# Autodesk Inventor assembly: ABD_Version_0.1_leftleg
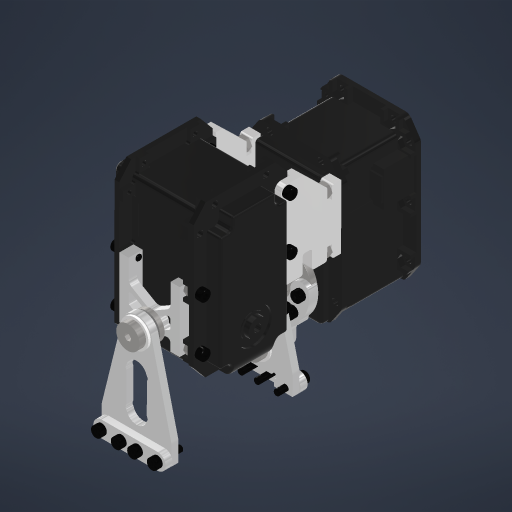
[picture p0: Inventor's stored thumbnail of the model, 512x512]
Saved by Autodesk Inventor 2024.3 (Build 283343000, 343)
## iProperties
Created: 2024-01-23
Part Number: ABD_Version_0.1_leftleg
Document SubType Name: Assembly
Designer: ASUS
Mass: 357.136 g
Surface Area: 604.848 cm^2
Volume: 181.423 cm^3
Density: 1.96853 g/cm^3
Author: ASUS
## Documents named in this file (19)
- C:\Users\ASUS\Desktop\test\v4_Frame\ABD_V4_Left_OP.iam
- C:\Users\ASUS\Desktop\test\v4_Frame\ABD_MX_64_Roll_Fixation_Set.iam
- C:\Users\ASUS\Desktop\test\v4_Frame\ABD_Slider_Set_v4.iam
- C:\Users\ASUS\Desktop\test\v1_Frame\MISUMI\C-WSSA12-4-2.ipt
- C:\Users\ASUS\Desktop\test\v4_Frame\Roll_Fixation_Frame_Back.ipt
- C:\Users\ASUS\Desktop\test\v4_Frame\hip joint fix washer.ipt
- C:\Users\ASUS\Desktop\test\Screw_Set\hip_joint_fix_washer_10mm_Set.iam
- C:\Users\ASUS\Desktop\test\v4_Frame\Front_Frame_Fixer_v2.iam
- C:\Users\ASUS\Desktop\test\ROBOTIS(Inventor 2024 ver.)\DXL\MX-64T.ipt
- C:\Users\ASUS\Desktop\test\v2_Frame\MISUMI\DBSY4-5-8.ipt
- C:\Users\ASUS\Desktop\test\v4_Frame\Dynamixel Vertical fixation.ipt
- C:\Users\ASUS\Desktop\test\v4_Frame\Dynamixel Vertical fixation_MIR.ipt
- C:\Users\ASUS\Desktop\test\v1_Frame\MISUMI\SLBNR2_5.ipt
- C:\Users\ASUS\Desktop\test\v4_Frame\MISUMI\TT-0612-05.ipt
- C:\Users\ASUS\Desktop\test\v4_Frame\MISUMI\LED-0605.ipt
- C:\Users\ASUS\Desktop\test\v4_Frame\MISUMI\DBB4-6-6.ipt
- C:\Users\ASUS\Desktop\test\v4_Frame\MISUMI\DBGS4-5-8.ipt
- C:\Users\ASUS\Desktop\test\Screw_Set\Roll_Fixation_Frame_8mm_Set.iam
- C:\Users\ASUS\Desktop\test\Screw_Set\Roll_Fixation_Frame_8mm_Set_Backside.iam
## Components (26 placed, 18 different names)
1. hip joint fix washer:1 — 삽입:64
2. hip joint fix washer:2 — 삽입:47, 메이트:29
3. hip_joint_fix_washer_10mm_Set:1 [sub-assembly] — 메이트:39
4. hip_joint_fix_washer_10mm_Set:2 [sub-assembly] — 메이트:29, 메이트:43
5. Front_Frame_Fixer_v2:1 [sub-assembly] — 삽입:46, 삽입:63, 삽입:73
6. DBSY4-5-8:1 — 삽입:73
7. ABD_MX_64_Roll_Fixation_Set:2 [sub-assembly] — 각도:3, 플러쉬:1, 삽입:46, 삽입:52, 삽입:71, 메이트:45, 삽입:72, 메이트:46
8. MX-64T:1 — 삽입:43, 각도:3, 플러쉬:1, 삽입:61, 메이트:35, 삽입:62, 메이트:36, 각도:13
9. ABD_Slider_Set_v4:2 [sub-assembly] — 삽입:43, 삽입:69
10. Roll_Fixation_Frame_Back:3 — 삽입:47, 메이트:43, 삽입:68, 메이트:44, 각도:13
11. Front_Frame_Fixer_v2:2 [sub-assembly] — 삽입:52, 삽입:68, 삽입:70
12. Dynamixel Vertical fixation:2 — 삽입:61, 메이트:35, 메이트:47, 메이트:48
13. Dynamixel Vertical fixation_MIR:2 — 삽입:62, 메이트:36
14. SLBNR2_5:5
15. SLBNR2_5:6
16. SLBNR2_5:7
17. SLBNR2_5:8
18. Roll_Fixation_Frame_Back:4 — 삽입:63, 메이트:39, 삽입:64
19. C-WSSA12-4-2:3 — 삽입:69
20. TT-0612-05:1
21. TT-0612-05:2
22. LED-0605:1 — 메이트:44
23. DBB4-6-6:1
24. DBGS4-5-8:1 — 삽입:70
25. Roll_Fixation_Frame_8mm_Set:1 [sub-assembly] — 삽입:71, 메이트:45
26. Roll_Fixation_Frame_8mm_Set_Backside:1 [sub-assembly] — 삽입:72, 메이트:46, 메이트:47, 메이트:48
## Relationships (46: Insert 23, Mate 16, Angle 6, Flush 1)
- [Insert]: hip joint fix washer:1 ↔ hip_joint_fix_washer_10mm_Set:1
- [Mate]: hip joint fix washer:1 ↔ hip_joint_fix_washer_10mm_Set:1
- [Insert]: hip joint fix washer:2 ↔ hip_joint_fix_washer_10mm_Set:2
- [Mate]: hip joint fix washer:2 ↔ hip_joint_fix_washer_10mm_Set:2
- [Mate]: hip_joint_fix_washer_10mm_Set:1 ↔ hip_joint_fix_washer_10mm_Set:2
- [Mate]: hip_joint_fix_washer_10mm_Set:1 ↔ hip_joint_fix_washer_10mm_Set:2
- 삽입:43 [Insert] (0.5 mm): MX-64T:1 ↔ ABD_Slider_Set_v4:2
- 각도:3 [Angle] (0 deg): ABD_MX_64_Roll_Fixation_Set:2 ↔ MX-64T:1
- 플러쉬:1 [Flush] (-3.1 mm): ABD_MX_64_Roll_Fixation_Set:2 ↔ MX-64T:1
- 삽입:46 [Insert]: Front_Frame_Fixer_v2:1 ↔ ABD_MX_64_Roll_Fixation_Set:2
- 삽입:47 [Insert]: hip joint fix washer:2 ↔ Roll_Fixation_Frame_Back:3
- 메이트:29 [Mate]: hip joint fix washer:2 ↔ hip_joint_fix_washer_10mm_Set:2
- 삽입:52 [Insert]: ABD_MX_64_Roll_Fixation_Set:2 ↔ Front_Frame_Fixer_v2:2
- [Insert]: Dynamixel Vertical fixation:2 ↔ SLBNR2_5:5
- [Insert]: Dynamixel Vertical fixation:2 ↔ SLBNR2_5:6
- [Insert]: Dynamixel Vertical fixation_MIR:2 ↔ SLBNR2_5:8
- [Insert]: Dynamixel Vertical fixation_MIR:2 ↔ SLBNR2_5:7
- [Angle] (0 deg): Dynamixel Vertical fixation_MIR:2 ↔ SLBNR2_5:7
- [Angle] (0 deg): Dynamixel Vertical fixation_MIR:2 ↔ SLBNR2_5:8
- [Angle] (0 deg): Dynamixel Vertical fixation:2 ↔ SLBNR2_5:5
- [Angle] (0 deg): Dynamixel Vertical fixation:2 ↔ SLBNR2_5:6
- 삽입:61 [Insert]: MX-64T:1 ↔ Dynamixel Vertical fixation:2
- 메이트:35 [Mate]: MX-64T:1 ↔ Dynamixel Vertical fixation:2
- 삽입:62 [Insert]: MX-64T:1 ↔ Dynamixel Vertical fixation_MIR:2
- 메이트:36 [Mate]: MX-64T:1 ↔ Dynamixel Vertical fixation_MIR:2
- 삽입:63 [Insert]: Front_Frame_Fixer_v2:1 ↔ Roll_Fixation_Frame_Back:4
- 메이트:39 [Mate]: hip_joint_fix_washer_10mm_Set:1 ↔ Roll_Fixation_Frame_Back:4
- 삽입:64 [Insert]: hip joint fix washer:1 ↔ Roll_Fixation_Frame_Back:4
- [Insert]: C-WSSA12-4-2:3 ↔ TT-0612-05:1
- [Insert]: TT-0612-05:1 ↔ LED-0605:1
- [Mate]: TT-0612-05:2 ↔ LED-0605:1
- [Mate]: TT-0612-05:2 ↔ LED-0605:1
- [Insert]: C-WSSA12-4-2:3 ↔ DBB4-6-6:1
- 메이트:43 [Mate]: hip_joint_fix_washer_10mm_Set:2 ↔ Roll_Fixation_Frame_Back:3
- 삽입:68 [Insert]: Roll_Fixation_Frame_Back:3 ↔ Front_Frame_Fixer_v2:2
- 삽입:69 [Insert]: ABD_Slider_Set_v4:2 ↔ C-WSSA12-4-2:3
- 메이트:44 [Mate]: Roll_Fixation_Frame_Back:3 ↔ LED-0605:1
- 삽입:70 [Insert]: Front_Frame_Fixer_v2:2 ↔ DBGS4-5-8:1
- 삽입:71 [Insert]: ABD_MX_64_Roll_Fixation_Set:2 ↔ Roll_Fixation_Frame_8mm_Set:1
- 메이트:45 [Mate]: ABD_MX_64_Roll_Fixation_Set:2 ↔ Roll_Fixation_Frame_8mm_Set:1
- 삽입:72 [Insert]: ABD_MX_64_Roll_Fixation_Set:2 ↔ Roll_Fixation_Frame_8mm_Set_Backside:1
- 메이트:46 [Mate]: ABD_MX_64_Roll_Fixation_Set:2 ↔ Roll_Fixation_Frame_8mm_Set_Backside:1
- 메이트:47 [Mate]: Dynamixel Vertical fixation:2 ↔ Roll_Fixation_Frame_8mm_Set_Backside:1
- 메이트:48 [Mate]: Dynamixel Vertical fixation:2 ↔ Roll_Fixation_Frame_8mm_Set_Backside:1
- 각도:13 [Angle] (0 deg): MX-64T:1 ↔ Roll_Fixation_Frame_Back:3
- 삽입:73 [Insert]: Front_Frame_Fixer_v2:1 ↔ DBSY4-5-8:1
## Named parameters: d1061_d1053 = 0 mm, d1062_d1054 = 0 mm, d1063_d1055 = 0 mm, d1064_d1056 = 0 mm, d1065_d1057 = 0 deg, d1066_d1058 = 0 deg, d1067_d1059 = 0 deg, d1068_d1060 = 0 deg
